# Autodesk Inventor assembly: Custom Lift
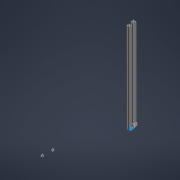
[picture p0: Inventor's stored thumbnail of the model, 180x180]
Saved by Autodesk Inventor 2022 (Build 260153000, 153)
## iProperties
Part Number: Custom Lift
Document SubType Name: Assembly
Designer: izack
Author: izack
## Documents named in this file (4)
- D:\Robotics\ComputerAidedDesign\2021-22\FTC\#12456 Big Red\Verical lift\Custom Lift\Custom Lift.iam
- D:\Robotics\ComputerAidedDesign\2021-22\FTC\#12456 Big Red\Verical lift\Custom Lift\15mm Extrusion - 420mm - 90° Ends.ipt
- D:\Robotics\ComputerAidedDesign\2021-22\FTC\#12456 Big Red\Verical lift\Custom Lift\8mm x 12mm x 3.5mm Flanged Bearing - 10 Pack.ipt
- D:\Robotics\ComputerAidedDesign\2021-22\FTC\#12456 Big Red\Verical lift\Custom Lift\Stationary Bracket.ipt
## Components (7 placed, 3 different names)
1. 15mm Extrusion - 420mm - 90° Ends:1 — Mate:2, Flush:1, Tangent:1, Tangent:2, Tangent:3
2. 8mm x 12mm x 3.5mm Flanged Bearing - 10 Pack:1
3. 8mm x 12mm x 3.5mm Flanged Bearing - 10 Pack:2
4. 8mm x 12mm x 3.5mm Flanged Bearing - 10 Pack:3 — Mate:5, Tangent:3
5. 8mm x 12mm x 3.5mm Flanged Bearing - 10 Pack:4 — Mate:5, Tangent:1, Tangent:2
6. 15mm Extrusion - 420mm - 90° Ends:2 — Mate:1, Mate:2, Flush:1, Mate:6, Mate:7, Flush:2
7. Stationary Bracket:1 — Mate:6, Mate:7, Flush:2
## Relationships (10: Mate 5, Tangent 3, Flush 2)
- Mate:1: 15mm Extrusion - 420mm - 90° Ends:2
- Mate:2 (4 mm): 15mm Extrusion - 420mm - 90° Ends:1 ↔ 15mm Extrusion - 420mm - 90° Ends:2
- Flush:1: 15mm Extrusion - 420mm - 90° Ends:1 ↔ 15mm Extrusion - 420mm - 90° Ends:2
- Mate:5: 8mm x 12mm x 3.5mm Flanged Bearing - 10 Pack:3 ↔ 8mm x 12mm x 3.5mm Flanged Bearing - 10 Pack:4
- Tangent:1: 15mm Extrusion - 420mm - 90° Ends:1 ↔ 8mm x 12mm x 3.5mm Flanged Bearing - 10 Pack:4
- Tangent:2: 15mm Extrusion - 420mm - 90° Ends:1 ↔ 8mm x 12mm x 3.5mm Flanged Bearing - 10 Pack:4
- Tangent:3: 15mm Extrusion - 420mm - 90° Ends:1 ↔ 8mm x 12mm x 3.5mm Flanged Bearing - 10 Pack:3
- Mate:6: 15mm Extrusion - 420mm - 90° Ends:2 ↔ Stationary Bracket:1
- Mate:7: 15mm Extrusion - 420mm - 90° Ends:2 ↔ Stationary Bracket:1
- Flush:2: 15mm Extrusion - 420mm - 90° Ends:2 ↔ Stationary Bracket:1
